# Autodesk Inventor assembly: 4x1inTractionWheel.1111-2016
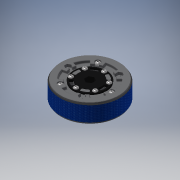
[picture p0: Inventor's stored thumbnail of the model, 180x180]
Saved by Autodesk Inventor 2016 (Build 200138000, 138)
## iProperties
Created: 2016-11-21
Part Number: 4x1inTractionWheel.1111-2016
Document SubType Name: Assembly
Designer: 589013
Mass: 204.905 g
Surface Area: 955.392 cm^2
Volume: 153.616 cm^3
Density: 1.33387 g/cm^3
Author: 589013
## Documents named in this file (9)
- C:\Users\smiku\GrabCAD\Power Hawks CAD\VEXpro Resources\Wheels\4 inch\4x1inTractionWheel-1111-2016.iam
- C:\Users\smiku\GrabCAD\Power Hawks CAD\VEXpro Resources\Wheels\Wheel Parts\4InchWheelEnd-1111-2016.ipt
- C:\Users\smiku\GrabCAD\Power Hawks CAD\VEXpro Resources\Fasteners\Standoffs\Standoff0.75in-1111-2016.ipt
- C:\Users\smiku\GrabCAD\Power Hawks CAD\VEXpro Resources\Fasteners\Screws\Screw8-32x1.25in-1111-2016.ipt
- C:\Users\smiku\GrabCAD\Power Hawks CAD\VEXpro Resources\Fasteners\Nuts\Nut8-32Nylock-1111-2016.ipt
- C:\Users\smiku\GrabCAD\Power Hawks CAD\VEXpro Resources\Versa Motion\VersaHub(0.5inHex)-1111-2016.ipt
- C:\Users\smiku\GrabCAD\Power Hawks CAD\VEXpro Resources\Versa Motion\VersaHub(0.5inHex,Plastic)-1111-2016.ipt
- C:\Users\smiku\GrabCAD\Power Hawks CAD\VEXpro Resources\Fasteners\Screws\Screw8-32x0.5in-1111-2016.ipt
- C:\Users\smiku\GrabCAD\Power Hawks CAD\VEXpro Resources\Wheels\Wheel Parts\4InchRoughTopTread(1inWidth)-1111-2017.ipt
## Components (29 placed, 8 different names)
1. 4InchWheelEnd-1111-2016:1 — Rotational:1, Angle:1, Rotational:2, Rotational:3, Rotational:4, Rotational:5, Rotational:6, Angle:2, Angle:3, Angle:4, Rotational:9, Rotational:10
2. 4InchWheelEnd-1111-2016:2 — Rotational:2, Rotational:3, Insert:1, Insert:2, Insert:3, Rotational:7, Rotational:8, Rigid:1
3. Screw8-32x1.25in-1111-2016:1 — Insert:1
4. Screw8-32x1.25in-1111-2016:2 — Insert:2
5. Screw8-32x1.25in-1111-2016:3 — Insert:3
6. Nut8-32Nylock-1111-2016:1 — Rotational:6, Angle:2
7. Nut8-32Nylock-1111-2016:2 — Rotational:5, Angle:4
8. Nut8-32Nylock-1111-2016:3 — Rotational:4, Angle:3
9. VersaHub(0.5inHex)-1111-2016:1 — Rotational:7, Rotational:8, Insert:4, Insert:5, Insert:6, Insert:7, Insert:8, Insert:9
10. VersaHub(0.5inHex,Plastic)-1111-2016:1 — Rotational:9, Rotational:10, Insert:10, Insert:11, Insert:12, Insert:13, Insert:14, Insert:15
11. Screw8-32x0.5in-1111-2016:1 — Insert:4
12. Screw8-32x0.5in-1111-2016:2 — Insert:6
13. Screw8-32x0.5in-1111-2016:3 — Insert:5
14. Screw8-32x0.5in-1111-2016:4 — Insert:7
15. Screw8-32x0.5in-1111-2016:5 — Insert:8
16. Screw8-32x0.5in-1111-2016:6 — Insert:9
17. Screw8-32x0.5in-1111-2016:7 — Insert:10
18. Screw8-32x0.5in-1111-2016:8 — Insert:11
19. Screw8-32x0.5in-1111-2016:9 — Insert:13
20. Screw8-32x0.5in-1111-2016:10 — Insert:14
21. Screw8-32x0.5in-1111-2016:11 — Insert:12
22. Screw8-32x0.5in-1111-2016:12 — Insert:15
23. 4InchRoughTopTread(1inWidth)-1111-2017:1 — Rigid:1
24. Standoff0.75in-1111-2016:1 — Rotational:1, Angle:1
25. Standoff0.75in-1111-2016:2
26. Standoff0.75in-1111-2016:3
27. Standoff0.75in-1111-2016:4
28. Standoff0.75in-1111-2016:5
29. Standoff0.75in-1111-2016:6
## Component patterns: (6 elements, first: Standoff0.75in-1111-2016:1)
## Relationships (30: Insert 15, RevoluteJoint 10, Angle 4, WeldJoint 1)
- Rotational:1 [RevoluteJoint]: 4InchWheelEnd-1111-2016:1 ↔ Standoff0.75in-1111-2016:1
- Angle:1 (0 deg): 4InchWheelEnd-1111-2016:1 ↔ Standoff0.75in-1111-2016:1
- Rotational:2 [RevoluteJoint]: 4InchWheelEnd-1111-2016:1 ↔ 4InchWheelEnd-1111-2016:2
- Rotational:3 [RevoluteJoint]: 4InchWheelEnd-1111-2016:1 ↔ 4InchWheelEnd-1111-2016:2
- Insert:1: 4InchWheelEnd-1111-2016:2 ↔ Screw8-32x1.25in-1111-2016:1
- Insert:2: 4InchWheelEnd-1111-2016:2 ↔ Screw8-32x1.25in-1111-2016:2
- Insert:3: 4InchWheelEnd-1111-2016:2 ↔ Screw8-32x1.25in-1111-2016:3
- Rotational:4 [RevoluteJoint]: 4InchWheelEnd-1111-2016:1 ↔ Nut8-32Nylock-1111-2016:3
- Rotational:5 [RevoluteJoint]: 4InchWheelEnd-1111-2016:1 ↔ Nut8-32Nylock-1111-2016:2
- Rotational:6 [RevoluteJoint]: 4InchWheelEnd-1111-2016:1 ↔ Nut8-32Nylock-1111-2016:1
- Angle:2 (0 deg): 4InchWheelEnd-1111-2016:1 ↔ Nut8-32Nylock-1111-2016:1
- Angle:3 (0 deg): 4InchWheelEnd-1111-2016:1 ↔ Nut8-32Nylock-1111-2016:3
- Angle:4 (0 deg): 4InchWheelEnd-1111-2016:1 ↔ Nut8-32Nylock-1111-2016:2
- Rotational:7 [RevoluteJoint]: 4InchWheelEnd-1111-2016:2 ↔ VersaHub(0.5inHex)-1111-2016:1
- Rotational:8 [RevoluteJoint]: 4InchWheelEnd-1111-2016:2 ↔ VersaHub(0.5inHex)-1111-2016:1
- Rotational:9 [RevoluteJoint]: 4InchWheelEnd-1111-2016:1 ↔ VersaHub(0.5inHex,Plastic)-1111-2016:1
- Rotational:10 [RevoluteJoint]: 4InchWheelEnd-1111-2016:1 ↔ VersaHub(0.5inHex,Plastic)-1111-2016:1
- Insert:4: VersaHub(0.5inHex)-1111-2016:1 ↔ Screw8-32x0.5in-1111-2016:1
- Insert:5: VersaHub(0.5inHex)-1111-2016:1 ↔ Screw8-32x0.5in-1111-2016:3
- Insert:6: VersaHub(0.5inHex)-1111-2016:1 ↔ Screw8-32x0.5in-1111-2016:2
- Insert:7: VersaHub(0.5inHex)-1111-2016:1 ↔ Screw8-32x0.5in-1111-2016:4
- Insert:8: VersaHub(0.5inHex)-1111-2016:1 ↔ Screw8-32x0.5in-1111-2016:5
- Insert:9: VersaHub(0.5inHex)-1111-2016:1 ↔ Screw8-32x0.5in-1111-2016:6
- Insert:10: VersaHub(0.5inHex,Plastic)-1111-2016:1 ↔ Screw8-32x0.5in-1111-2016:7
- Insert:11: VersaHub(0.5inHex,Plastic)-1111-2016:1 ↔ Screw8-32x0.5in-1111-2016:8
- Insert:12: VersaHub(0.5inHex,Plastic)-1111-2016:1 ↔ Screw8-32x0.5in-1111-2016:11
- Insert:13: VersaHub(0.5inHex,Plastic)-1111-2016:1 ↔ Screw8-32x0.5in-1111-2016:9
- Insert:14: VersaHub(0.5inHex,Plastic)-1111-2016:1 ↔ Screw8-32x0.5in-1111-2016:10
- Insert:15: VersaHub(0.5inHex,Plastic)-1111-2016:1 ↔ Screw8-32x0.5in-1111-2016:12
- Rigid:1 [WeldJoint]: 4InchWheelEnd-1111-2016:2 ↔ 4InchRoughTopTread(1inWidth)-1111-2017:1
